# Autodesk Inventor assembly: gearbox
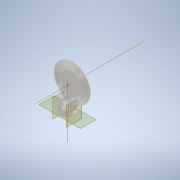
[picture p0: Inventor's stored thumbnail of the model, 180x180]
Saved by Autodesk Inventor 2020 (Build 240168000, 168)
## iProperties
Created: 2019-06-21
Part Number: gearbox
Document SubType Name: Assembly
Designer: User
Author: User
## Documents named in this file (2)
- F:\Library\Documents\Project_quick_temp\Gear_box_3\gearbox.iam
- F:\Library\Documents\Project_quick_temp\Gear_box_3\gearbox\设计加速器\锥齿轮1.iam
## Components (1 placed, 1 different names)
1. 锥齿轮:1 [sub-assembly] — 表面齐平:1
## Relationships (1: Flush 1)
- 表面齐平:1 [Flush] (-2.5 mm): 锥齿轮:1
